# Autodesk Inventor assembly: LimitSwitchAssembly
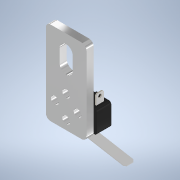
[picture p0: Inventor's stored thumbnail of the model, 180x180]
Saved by Autodesk Inventor 2020.4 (Build 244396010, 396A)
## iProperties
Created: 2021-10-18
Part Number: LimitSwitchAssembly
Document SubType Name: Assembly
Designer: justi
Author: justi
## Documents named in this file (3)
- D:\UQ Engineering\2021 ~ 5th Year\Semester 2\METR4911-THESIS\FarmBot CAD\FarmBotV1\LimitSwitchAssembly.iam
- D:\UQ Engineering\2021 ~ 5th Year\Semester 2\METR4911-THESIS\FarmBot CAD\FarmBotV1\limitswitch.ipt
- D:\UQ Engineering\2021 ~ 5th Year\Semester 2\METR4911-THESIS\FarmBot CAD\FarmBotV1\LimitSwitchMount.ipt
## Components (2 placed, 2 different names)
1. limitswitch:1 — Mate:1, Mate:2, Mate:3
2. LimitSwitchMount:1 — Mate:1, Mate:2, Mate:3
## Relationships (3: Mate 3)
- Mate:1: limitswitch:1 ↔ LimitSwitchMount:1
- Mate:2: limitswitch:1 ↔ LimitSwitchMount:1
- Mate:3: limitswitch:1 ↔ LimitSwitchMount:1
